# Autodesk Inventor assembly: BungaSign-Biggerv2
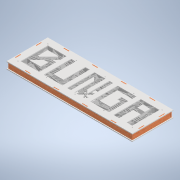
[picture p0: Inventor's stored thumbnail of the model, 180x180]
Saved by Autodesk Inventor 2022 (Build 260153000, 153)
## iProperties
Created: 2022-08-17
Part Number: BungaSign-Biggerv2
Document SubType Name: Assembly
Designer: incep
Author: incep
## Documents named in this file (13)
- C:\Projects\BungaSign\BungaSign-Biggerv2.iam
- C:\Projects\BungaSign\BungaSign-Bigger.ipt
- C:\Projects\BungaSign\BungaSign-Bigger-Layer1v2.ipt
- C:\Projects\BungaSign\BungaSign-Bigger-Layer2v2.ipt
- C:\Projects\BungaSign\BungaSign-Bigger-Layer3v2.ipt
- C:\Projects\BungaSign\BungaSign-Bigger-Layer4v2.ipt
- C:\Projects\BungaSign\BungaSign-Bigger-Layer5v2.ipt
- C:\Projects\BungaSign\BungaSign-Bigger-Layer6v2.ipt
- C:\Projects\BungaSign\BungaSign-Bigger-Layer7v2.ipt
- C:\Projects\BungaSign\BungaSign-Bigger-Back.ipt
- C:\Projects\BungaSign\BungaSign-Bigger-Sides-TopBottom.ipt
- C:\Projects\BungaSign\BungaSign-Bigger-Sides-Left.ipt
- C:\Projects\BungaSign\BungaSign-Bigger-Sides-Right.ipt
## Components (13 placed, 12 different names)
1. BungaSign-Bigger:1 — Flush:1, Mate:1, Mate:2, Mate:3, Mate:6, Mate:8, Mate:9, Mate:12, Mate:15, Mate:17, Mate:18, Mate:20, Mate:21, Mate:23, Mate:24, Flush:2, Mate:25, Mate:26, Flush:3, Mate:27, Mate:28, Flush:4, Mate:29, Mate:30, Flush:5, Mate:31, Mate:32
2. BungaSign-Bigger-Layer1v2:1 — Mate:1, Mate:2, Mate:3, Mate:4, Mate:5
3. BungaSign-Bigger-Layer2v2:1 — Mate:4, Mate:5, Mate:6, Mate:7
4. BungaSign-Bigger-Layer3v2:1 — Mate:7, Mate:8, Mate:9, Mate:10, Mate:11
5. BungaSign-Bigger-Layer4v2:1 — Mate:10, Mate:11, Mate:12, Mate:13, Mate:14
6. BungaSign-Bigger-Layer5v2:1 — Mate:13, Mate:14, Mate:15, Mate:16
7. BungaSign-Bigger-Layer6v2:1 — Mate:16, Mate:17, Mate:18, Mate:19
8. BungaSign-Bigger-Layer7v2:1 — Mate:19, Mate:20, Mate:21, Mate:22
9. BungaSign-Bigger-Back:1 — Mate:22, Mate:23, Mate:24
10. BungaSign-Bigger-Sides-TopBottom:1 — Flush:2, Mate:25, Mate:26
11. BungaSign-Bigger-Sides-TopBottom:2 — Flush:3, Mate:27, Mate:28
12. BungaSign-Bigger-Sides-Left:1 — Flush:4, Mate:29, Mate:30
13. BungaSign-Bigger-Sides-Right:1 — Flush:5, Mate:31, Mate:32
## Relationships (37: Mate 32, Flush 5)
- Flush:1: BungaSign-Bigger:1
- Mate:1: BungaSign-Bigger:1 ↔ BungaSign-Bigger-Layer1v2:1
- Mate:2: BungaSign-Bigger:1 ↔ BungaSign-Bigger-Layer1v2:1
- Mate:3: BungaSign-Bigger:1 ↔ BungaSign-Bigger-Layer1v2:1
- Mate:4: BungaSign-Bigger-Layer1v2:1 ↔ BungaSign-Bigger-Layer2v2:1
- Mate:5: BungaSign-Bigger-Layer1v2:1 ↔ BungaSign-Bigger-Layer2v2:1
- Mate:6: BungaSign-Bigger:1 ↔ BungaSign-Bigger-Layer2v2:1
- Mate:7: BungaSign-Bigger-Layer2v2:1 ↔ BungaSign-Bigger-Layer3v2:1
- Mate:8: BungaSign-Bigger:1 ↔ BungaSign-Bigger-Layer3v2:1
- Mate:9: BungaSign-Bigger:1 ↔ BungaSign-Bigger-Layer3v2:1
- Mate:10: BungaSign-Bigger-Layer3v2:1 ↔ BungaSign-Bigger-Layer4v2:1
- Mate:11: BungaSign-Bigger-Layer3v2:1 ↔ BungaSign-Bigger-Layer4v2:1
- Mate:12: BungaSign-Bigger:1 ↔ BungaSign-Bigger-Layer4v2:1
- Mate:13: BungaSign-Bigger-Layer4v2:1 ↔ BungaSign-Bigger-Layer5v2:1
- Mate:14: BungaSign-Bigger-Layer4v2:1 ↔ BungaSign-Bigger-Layer5v2:1
- Mate:15: BungaSign-Bigger:1 ↔ BungaSign-Bigger-Layer5v2:1
- Mate:16: BungaSign-Bigger-Layer5v2:1 ↔ BungaSign-Bigger-Layer6v2:1
- Mate:17: BungaSign-Bigger:1 ↔ BungaSign-Bigger-Layer6v2:1
- Mate:18: BungaSign-Bigger:1 ↔ BungaSign-Bigger-Layer6v2:1
- Mate:19: BungaSign-Bigger-Layer6v2:1 ↔ BungaSign-Bigger-Layer7v2:1
- Mate:20: BungaSign-Bigger:1 ↔ BungaSign-Bigger-Layer7v2:1
- Mate:21: BungaSign-Bigger:1 ↔ BungaSign-Bigger-Layer7v2:1
- Mate:22: BungaSign-Bigger-Layer7v2:1 ↔ BungaSign-Bigger-Back:1
- Mate:23: BungaSign-Bigger:1 ↔ BungaSign-Bigger-Back:1
- Mate:24: BungaSign-Bigger:1 ↔ BungaSign-Bigger-Back:1
- Flush:2: BungaSign-Bigger:1 ↔ BungaSign-Bigger-Sides-TopBottom:1
- Mate:25: BungaSign-Bigger:1 ↔ BungaSign-Bigger-Sides-TopBottom:1
- Mate:26: BungaSign-Bigger:1 ↔ BungaSign-Bigger-Sides-TopBottom:1
- Flush:3: BungaSign-Bigger:1 ↔ BungaSign-Bigger-Sides-TopBottom:2
- Mate:27: BungaSign-Bigger:1 ↔ BungaSign-Bigger-Sides-TopBottom:2
- Mate:28: BungaSign-Bigger:1 ↔ BungaSign-Bigger-Sides-TopBottom:2
- Flush:4: BungaSign-Bigger:1 ↔ BungaSign-Bigger-Sides-Left:1
- Mate:29: BungaSign-Bigger:1 ↔ BungaSign-Bigger-Sides-Left:1
- Mate:30: BungaSign-Bigger:1 ↔ BungaSign-Bigger-Sides-Left:1
- Flush:5: BungaSign-Bigger:1 ↔ BungaSign-Bigger-Sides-Right:1
- Mate:31: BungaSign-Bigger:1 ↔ BungaSign-Bigger-Sides-Right:1
- Mate:32: BungaSign-Bigger:1 ↔ BungaSign-Bigger-Sides-Right:1
